# Autodesk Inventor assembly: HIN-61 BISAGRA (P1 MARCO)
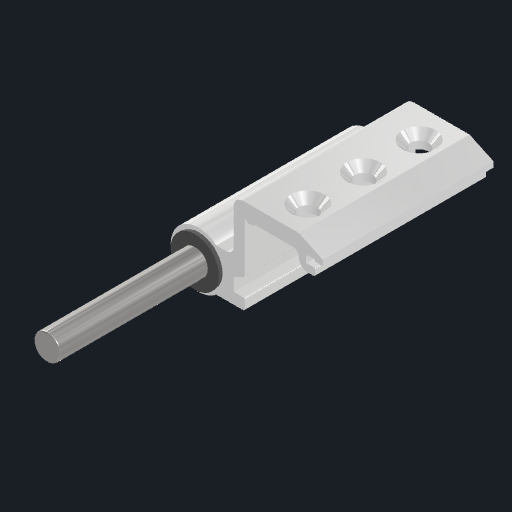
[picture p0: Inventor's stored thumbnail of the model, 512x512]
Saved by Autodesk Inventor 2025 (Build 290162000, 162)
## iProperties
Created: 2026-02-23
Part Number: HIN-61 BISAGRA (P1 MARCO)
Document SubType Name: Assembly
Designer: ROLANDO
Author: ROLANDO
## Documents named in this file (5)
- C:\Users\rolan\OneDrive\Documentos\Inventor\Projects\CARPINTERIA ALUMINIO\PUERTAS Y VENTANAS\ACCESORIOS\BISAGRAS\ENSAMBLES\HIN-61 BISAGRA (P1 MARCO-PASADOR).iam
- HIN-61 BISAGRA (P1 MARCO-PASADOR).iam
- C:\Users\rolan\OneDrive\Documentos\Inventor\Projects\CARPINTERIA ALUMINIO\PUERTAS Y VENTANAS\ACCESORIOS\BISAGRAS\PIEZAS\HIN-61 BISAGRA\HIN-61 BISAGRA (P1 MARCO).ipt
- C:\Users\rolan\OneDrive\Documentos\Inventor\Projects\CARPINTERIA ALUMINIO\PUERTAS Y VENTANAS\ACCESORIOS\BISAGRAS\PIEZAS\HIN-61 BISAGRA\HIN-61 BISAGRA (BUJE PLASTICO).ipt
- C:\Users\rolan\OneDrive\Documentos\Inventor\Projects\CARPINTERIA ALUMINIO\PUERTAS Y VENTANAS\ACCESORIOS\BISAGRAS\PIEZAS\HIN-61 BISAGRA\HIN-61 BISAGRA (PASADOR).ipt
## Components (3 placed, 3 different names)
1. HIN-61 BISAGRA (P1 MARCO):1 — Coincidencia:1, Coincidencia:2, Coincidencia:3
2. HIN-61 BISAGRA (BUJE PLASTICO):1 — Coincidencia:1, Coincidencia:2, Coincidencia:3, Insertar:1
3. HIN-61 BISAGRA (PASADOR):1 — Insertar:1
## Relationships (4: Mate 3, Insert 1)
- Coincidencia:1 [Mate]: HIN-61 BISAGRA (P1 MARCO):1 ↔ HIN-61 BISAGRA (BUJE PLASTICO):1
- Coincidencia:2 [Mate]: HIN-61 BISAGRA (P1 MARCO):1 ↔ HIN-61 BISAGRA (BUJE PLASTICO):1
- Coincidencia:3 [Mate]: HIN-61 BISAGRA (P1 MARCO):1 ↔ HIN-61 BISAGRA (BUJE PLASTICO):1
- Insertar:1 (-39.5 mm): HIN-61 BISAGRA (BUJE PLASTICO):1 ↔ HIN-61 BISAGRA (PASADOR):1
